# Autodesk Inventor assembly: mill_assembly
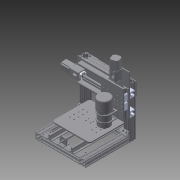
[picture p0: Inventor's stored thumbnail of the model, 180x180]
Saved by Autodesk Inventor 2014 (Build 180170000, 170)
## iProperties
Created: 2014-08-08
Part Number: mill_assembly
Document SubType Name: Assembly
Designer: Matthew
Author: Matthew
## Documents named in this file (29)
- C:\Users\Matthew\Documents\GitHub\CNC Mill\mill_assembly.iam
- C:\Users\Matthew\Documents\GitHub\CNC Mill\Imported Components\8020-2040\Assembly2.iam
- C:\Users\Matthew\Documents\GitHub\CNC Mill\8020\2020.ipt
- C:\Users\Matthew\Documents\GitHub\CNC Mill\8020\2020_18in.ipt
- C:\Users\Matthew\Documents\GitHub\CNC Mill\plate_4127.ipt
- C:\Users\Matthew\Documents\GitHub\CNC Mill\8020\gusset_4138.ipt
- C:\Users\Matthew\Documents\GitHub\CNC Mill\8020\gusset_4134.ipt
- C:\Users\Matthew\Documents\GitHub\CNC Mill\mic6_plate.ipt
- C:\Users\Matthew\Documents\GitHub\CNC Mill\1605\1605_400mm.ipt
- C:\Users\Matthew\Documents\GitHub\CNC Mill\1605\1605_ballnut.ipt
- C:\Users\Matthew\Documents\GitHub\CNC Mill\y_axis_mounting_plate.ipt
- C:\Users\Matthew\Documents\GitHub\CNC Mill\nema23_motor_mount.ipt
- C:\Users\Matthew\Documents\GitHub\CNC Mill\fk12.ipt
- C:\Users\Matthew\Documents\GitHub\CNC Mill\sbr\sbr20\SBR20UU.iam
- C:\Users\Matthew\Documents\GitHub\CNC Mill\6.35x10mm_coupler.ipt
- C:\Users\Matthew\Documents\GitHub\CNC Mill\sbr\sbr20\sbr20_400mm.ipt
- C:\Users\Matthew\Documents\GitHub\CNC Mill\HD16.ipt
- C:\Users\Matthew\Documents\GitHub\CNC Mill\nema23_HS8630.ipt
- C:\Users\Matthew\Documents\GitHub\CNC Mill\sbr\sbr20\sbr20_210mm.ipt
- C:\Users\Matthew\Documents\GitHub\CNC Mill\sbr\sbr20\sbr20_360mm.ipt
- C:\Users\Matthew\Documents\GitHub\CNC Mill\z-axis_mount_plate.ipt
- C:\Users\Matthew\Documents\GitHub\CNC Mill\1605\1605_200mm.ipt
- C:\Users\Matthew\Documents\GitHub\CNC Mill\y-axis_mount_plate.ipt
- C:\Users\Matthew\Documents\GitHub\CNC Mill\8020\2020_16in.ipt
- C:\Users\Matthew\Documents\GitHub\CNC Mill\router_plate.ipt
- C:\Users\Matthew\Documents\GitHub\CNC Mill\router_mount.ipt
- C:\Users\Matthew\Documents\GitHub\CNC Mill\1617evs.ipt
- C:\Users\Matthew\Documents\GitHub\CNC Mill\ff12_mount.ipt
- C:\Users\Matthew\Documents\GitHub\CNC Mill\ff12.ipt
## Components (67 placed, 28 different names)
1. Assembly2:1 [sub-assembly] — Mate:22, Mate:24, Mate:26, Mate:39, Mate:41, Mate:42, Mate:43, Mate:45, Mate:161, Flush:91, Flush:114, Flush:115, Mate:184, Flush:117, Flush:118, Mate:185
2. 2020_18in:1 — Mate:31, Mate:32, Mate:38, Mate:47, Mate:48, Mate:111, Flush:66, Mate:181, Flush:107, Flush:108, Flush:113
3. 2020_18in:2 — Mate:28, Mate:29, Mate:34, Mate:50, Mate:51, Flush:60, Flush:109, Flush:110, Mate:182
4. 2020:3 — Mate:46, Mate:49, Mate:115, Flush:63, Mate:116, Mate:127, Mate:128, Flush:111, Flush:112, Mate:183
5. 2020:4 — Mate:111, Flush:60, Mate:113, Mate:114, Flush:66, Flush:67, Flush:68, Flush:108, Flush:109, Flush:110, Mate:182, Flush:124, Mate:190
6. plate_4127:1 — Mate:39, Mate:41, Flush:119
7. gusset_4138:1 — Mate:22
8. gusset_4134:1 — Mate:28, Mate:29
9. gusset_4138:2 — Mate:24, Mate:26
10. gusset_4134:2 — Mate:31, Mate:32
11. gusset_4134:3 — Mate:34, Mate:113, Flush:61
12. gusset_4134:4 — Mate:38, Mate:114, Flush:62
13. plate_4127:2 — Mate:42, Mate:43, Mate:45, Flush:116
14. gusset_4134:5 — Mate:49, Mate:50, Mate:51
15. gusset_4134:6 — Mate:46, Mate:47, Mate:48, Flush:61, Flush:62
16. mic6_plate:1 — Flush:76, Flush:77, Mate:141
17. 1605_400mm:1 — Mate:98, Mate:100, Mate:108, Insert:2
18. 1605_ballnut:1 — Mate:108, Mate:133, Mate:134, Flush:75
19. y_axis_mounting_plate:1
20. nema23_motor_mount:1 — Mate:99, Mate:115, Flush:63, Mate:116, Mate:136, Mate:137
21. nema23_motor_mount:2 — Mate:153, Flush:86, Mate:154, Mate:155, Mate:156, Mate:157
22. 1605_ballnut:5
23. 1605_ballnut:6 — Mate:150, Mate:158, Flush:90, Mate:159
24. fk12:1 — Mate:98, Mate:99, Mate:100, Mate:137
25. nema23_motor_mount:3
26. fk12:3 — Mate:156, Mate:157
27. SBR20UU:1 [sub-assembly] — Mate:131, Flush:69, Flush:70, Flush:73, Mate:138, Mate:140, Flush:77, Mate:141
28. 6.35x10mm_coupler:1 — Insert:3, Insert:4
29. sbr20_400mm:1 — Mate:127, Flush:67, Mate:130
30. SBR20UU:2 [sub-assembly] — Mate:129, Mate:132, Flush:71, Flush:72, Mate:139
31. sbr20_400mm:2 — Flush:68, Mate:128, Mate:129
32. SBR20UU:3 [sub-assembly] — Mate:130, Mate:131, Flush:69, Flush:70, Flush:74, Flush:76
33. SBR20UU:4 [sub-assembly] — Mate:132, Flush:71, Flush:72, Flush:73, Flush:74
34. HD16:1 — Mate:133, Mate:134, Flush:75, Mate:138, Mate:139, Mate:140
35. nema23_HS8630:1 — Mate:135, Mate:136
36. 6.35x10mm_coupler:2 — Insert:2, Mate:135
37. sbr20_210mm:1 — Mate:143, Mate:149, Flush:82, Mate:168, Flush:104
38. sbr20_360mm:1 — Mate:162, Flush:92, Mate:165, Mate:178, Flush:106
39. SBR20UU:5 [sub-assembly] — Mate:143, Flush:78, Flush:79, Mate:144, Flush:84, Flush:85, Mate:160
40. SBR20UU:6 [sub-assembly] — Flush:78, Flush:79, Mate:144
41. sbr20_210mm:2 — Mate:148, Flush:83, Mate:169
42. SBR20UU:7 [sub-assembly] — Flush:84, Flush:85
43. SBR20UU:8 [sub-assembly]
44. z-axis_mount_plate:1 — Mate:148, Mate:149, Flush:82, Flush:83, Mate:153, Flush:86, Mate:167, Flush:102, Flush:103, Flush:104
45. 1605_200mm:1 — Mate:150, Insert:3
46. nema23_HS8630:2 — Mate:154, Mate:155, Insert:4
47. HD16:6 — Mate:158, Flush:90, Mate:159, Mate:160, Mate:168, Mate:169, Mate:186, Flush:120, Flush:121
48. y-axis_mount_plate:1 — Mate:161, Flush:91, Mate:162, Mate:163, Mate:177, Flush:106
49. sbr20_360mm:2 — Flush:92, Mate:163, Mate:164, Mate:179, Mate:188
50. SBR20UU:9 [sub-assembly] — Mate:164, Flush:95, Flush:96, Flush:99, Flush:101, Mate:167, Flush:103
51. SBR20UU:10 [sub-assembly] — Mate:165, Flush:95, Flush:96, Mate:166, Flush:97, Flush:98, Flush:102
52. SBR20UU:11 [sub-assembly] — Flush:99, Flush:100, Flush:101
53. SBR20UU:12 [sub-assembly] — Mate:166, Flush:97, Flush:98, Flush:100, Mate:180
54. nema23_motor_mount:4 — Mate:177
55. fk12:4 — Insert:8, Mate:188
56. 6.35x10mm_coupler:3
57. nema23_HS8630:3
58. 1605_400mm:2 — Mate:176, Insert:8
59. 1605_ballnut:7 — Mate:176
60. HD16:7 — Mate:178, Mate:179, Mate:180
61. 2020_16in:1 — Mate:181, Flush:107, Flush:111, Flush:112, Flush:113, Mate:183, Flush:114, Flush:115, Mate:184, Flush:116
62. 2020_16in:2 — Flush:117, Flush:118, Mate:185, Flush:119
63. router_plate:1 — Mate:186, Flush:120, Flush:121, Mate:187, Flush:122, Flush:123
64. router_mount:1 — Insert:7, Mate:187, Flush:122, Flush:123
65. 1617evs:1 — Insert:7
66. ff12_mount:1 — Flush:124, Mate:190, Insert:9
67. ff12:1 — Insert:9
## Relationships (153: Mate 88, Flush 58, Insert 7)
- Mate:22: Assembly2:1 ↔ gusset_4138:1
- Mate:24: Assembly2:1 ↔ gusset_4138:2
- Mate:26: Assembly2:1 ↔ gusset_4138:2
- Mate:28: 2020_18in:2 ↔ gusset_4134:1
- Mate:29: 2020_18in:2 ↔ gusset_4134:1
- Mate:31: 2020_18in:1 ↔ gusset_4134:2
- Mate:32: 2020_18in:1 ↔ gusset_4134:2
- Mate:34: 2020_18in:2 ↔ gusset_4134:3
- Mate:38: 2020_18in:1 ↔ gusset_4134:4
- Mate:39: Assembly2:1 ↔ plate_4127:1
- Mate:41: Assembly2:1 ↔ plate_4127:1
- Mate:42: Assembly2:1 ↔ plate_4127:2
- Mate:43: Assembly2:1 ↔ plate_4127:2
- Mate:45: Assembly2:1 ↔ plate_4127:2
- Mate:46: 2020:3 ↔ gusset_4134:6
- Mate:47: 2020_18in:1 ↔ gusset_4134:6
- Mate:48: 2020_18in:1 ↔ gusset_4134:6
- Mate:49: 2020:3 ↔ gusset_4134:5
- Mate:50: 2020_18in:2 ↔ gusset_4134:5
- Mate:51: 2020_18in:2 ↔ gusset_4134:5
- Mate:98: 1605_400mm:1 ↔ fk12:1
- Mate:99: nema23_motor_mount:1 ↔ fk12:1
- Mate:100: 1605_400mm:1 ↔ fk12:1
- Mate:108: 1605_400mm:1 ↔ 1605_ballnut:1
- Mate:111: 2020_18in:1 ↔ 2020:4
- Flush:60: 2020_18in:2 ↔ 2020:4
- Mate:113: 2020:4 ↔ gusset_4134:3
- Flush:61: gusset_4134:3 ↔ gusset_4134:6
- Mate:114: 2020:4 ↔ gusset_4134:4
- Flush:62: gusset_4134:4 ↔ gusset_4134:6
- Mate:115: 2020:3 ↔ nema23_motor_mount:1
- Flush:63: 2020:3 ↔ nema23_motor_mount:1
- Mate:116 (124.2695 mm): 2020:3 ↔ nema23_motor_mount:1
- Flush:66: 2020_18in:1 ↔ 2020:4
- Mate:127: 2020:3 ↔ sbr20_400mm:1
- Flush:67: 2020:4 ↔ sbr20_400mm:1
- Flush:68: 2020:4 ↔ sbr20_400mm:2
- Mate:128: 2020:3 ↔ sbr20_400mm:2
- Mate:129: SBR20UU:2 ↔ sbr20_400mm:2
- Mate:130: sbr20_400mm:1 ↔ SBR20UU:3
- Mate:131 (20 mm): SBR20UU:1 ↔ SBR20UU:3
- Flush:69: SBR20UU:1 ↔ SBR20UU:3
- Flush:70: SBR20UU:1 ↔ SBR20UU:3
- Mate:132 (20 mm): SBR20UU:2 ↔ SBR20UU:4
- Flush:71: SBR20UU:2 ↔ SBR20UU:4
- Flush:72: SBR20UU:2 ↔ SBR20UU:4
- Flush:73: SBR20UU:1 ↔ SBR20UU:4
- Flush:74: SBR20UU:3 ↔ SBR20UU:4
- Mate:133: 1605_ballnut:1 ↔ HD16:1
- Mate:134: 1605_ballnut:1 ↔ HD16:1
- Flush:75: 1605_ballnut:1 ↔ HD16:1
- Insert:2 (-12.5 mm): 1605_400mm:1 ↔ 6.35x10mm_coupler:2
- Mate:135: nema23_HS8630:1 ↔ 6.35x10mm_coupler:2
- Mate:136: nema23_motor_mount:1 ↔ nema23_HS8630:1
- Mate:137: nema23_motor_mount:1 ↔ fk12:1
- Mate:138 (42.3 mm): SBR20UU:1 ↔ HD16:1
- Mate:139 (42.3 mm): SBR20UU:2 ↔ HD16:1
- Mate:140 (-7.5 mm): SBR20UU:1 ↔ HD16:1
- Flush:76 (38.1 mm): mic6_plate:1 ↔ SBR20UU:3
- Flush:77 (-92.4052 mm): mic6_plate:1 ↔ SBR20UU:1
- Mate:141: mic6_plate:1 ↔ SBR20UU:1
- Mate:143: sbr20_210mm:1 ↔ SBR20UU:5
- Flush:78: SBR20UU:5 ↔ SBR20UU:6
- Flush:79: SBR20UU:5 ↔ SBR20UU:6
- Mate:144 (10 mm): SBR20UU:5 ↔ SBR20UU:6
- [Mate]: sbr20_210mm:2 ↔ SBR20UU:7
- [Flush]: SBR20UU:7 ↔ SBR20UU:8
- [Flush]: SBR20UU:7 ↔ SBR20UU:8
- [Mate] (10 mm): SBR20UU:7 ↔ SBR20UU:8
- Mate:148: sbr20_210mm:2 ↔ z-axis_mount_plate:1
- Mate:149: sbr20_210mm:1 ↔ z-axis_mount_plate:1
- Flush:82: sbr20_210mm:1 ↔ z-axis_mount_plate:1
- Flush:83: sbr20_210mm:2 ↔ z-axis_mount_plate:1
- Flush:84: SBR20UU:5 ↔ SBR20UU:7
- Flush:85: SBR20UU:5 ↔ SBR20UU:7
- Mate:150: 1605_ballnut:6 ↔ 1605_200mm:1
- Insert:3 (-12.5 mm): 6.35x10mm_coupler:1 ↔ 1605_200mm:1
- Mate:153: nema23_motor_mount:2 ↔ z-axis_mount_plate:1
- Flush:86: nema23_motor_mount:2 ↔ z-axis_mount_plate:1
- Mate:154: nema23_motor_mount:2 ↔ nema23_HS8630:2
- Mate:155: nema23_motor_mount:2 ↔ nema23_HS8630:2
- Insert:4 (-7 mm): 6.35x10mm_coupler:1 ↔ nema23_HS8630:2
- Mate:156: nema23_motor_mount:2 ↔ fk12:3
- Mate:157: nema23_motor_mount:2 ↔ fk12:3
- Mate:158: 1605_ballnut:6 ↔ HD16:6
- Flush:90: 1605_ballnut:6 ↔ HD16:6
- Mate:159: 1605_ballnut:6 ↔ HD16:6
- Mate:160 (-12.5 mm): SBR20UU:5 ↔ HD16:6
- Mate:161: Assembly2:1 ↔ y-axis_mount_plate:1
- Flush:91: Assembly2:1 ↔ y-axis_mount_plate:1
- Mate:162: sbr20_360mm:1 ↔ y-axis_mount_plate:1
- Flush:92: sbr20_360mm:1 ↔ sbr20_360mm:2
- Mate:163: y-axis_mount_plate:1 ↔ sbr20_360mm:2
- Mate:164: sbr20_360mm:2 ↔ SBR20UU:9
- Mate:165: sbr20_360mm:1 ↔ SBR20UU:10
- Flush:95: SBR20UU:9 ↔ SBR20UU:10
- Flush:96: SBR20UU:9 ↔ SBR20UU:10
- Mate:166 (60 mm): SBR20UU:10 ↔ SBR20UU:12
- Flush:97: SBR20UU:10 ↔ SBR20UU:12
- Flush:98: SBR20UU:10 ↔ SBR20UU:12
- Flush:99: SBR20UU:9 ↔ SBR20UU:11
- Flush:100: SBR20UU:11 ↔ SBR20UU:12
- Flush:101: SBR20UU:9 ↔ SBR20UU:11
- Mate:167: z-axis_mount_plate:1 ↔ SBR20UU:9
- Flush:102: z-axis_mount_plate:1 ↔ SBR20UU:10
- Flush:103: z-axis_mount_plate:1 ↔ SBR20UU:9
- Mate:168 (11 mm): sbr20_210mm:1 ↔ HD16:6
- Mate:169 (11 mm): sbr20_210mm:2 ↔ HD16:6
- Flush:104: sbr20_210mm:1 ↔ z-axis_mount_plate:1
- [Mate]: nema23_motor_mount:4 ↔ nema23_HS8630:3
- [Mate]: nema23_motor_mount:4 ↔ nema23_HS8630:3
- [Insert] (-7 mm): 6.35x10mm_coupler:3 ↔ nema23_HS8630:3
- [Mate]: nema23_motor_mount:4 ↔ fk12:4
- [Mate]: nema23_motor_mount:4 ↔ fk12:4
- [Mate]: 1605_ballnut:7 ↔ HD16:7
- [Flush]: 1605_ballnut:7 ↔ HD16:7
- [Mate]: 1605_ballnut:7 ↔ HD16:7
- Mate:176: 1605_400mm:2 ↔ 1605_ballnut:7
- Mate:177: y-axis_mount_plate:1 ↔ nema23_motor_mount:4
- Mate:178 (19.9 mm): sbr20_360mm:1 ↔ HD16:7
- Mate:179 (19.9 mm): sbr20_360mm:2 ↔ HD16:7
- Flush:106: sbr20_360mm:1 ↔ y-axis_mount_plate:1
- Mate:180 (12.5 mm): SBR20UU:12 ↔ HD16:7
- Mate:181: 2020_18in:1 ↔ 2020_16in:1
- Flush:107: 2020_18in:1 ↔ 2020_16in:1
- Flush:108: 2020_18in:1 ↔ 2020:4
- Flush:109: 2020_18in:2 ↔ 2020:4
- Flush:110: 2020_18in:2 ↔ 2020:4
- Mate:182: 2020_18in:2 ↔ 2020:4
- Flush:111: 2020:3 ↔ 2020_16in:1
- Flush:112: 2020:3 ↔ 2020_16in:1
- Flush:113: 2020_18in:1 ↔ 2020_16in:1
- Mate:183: 2020:3 ↔ 2020_16in:1
- Flush:114: Assembly2:1 ↔ 2020_16in:1
- Flush:115: Assembly2:1 ↔ 2020_16in:1
- Mate:184: Assembly2:1 ↔ 2020_16in:1
- Flush:116: plate_4127:2 ↔ 2020_16in:1
- Flush:117: Assembly2:1 ↔ 2020_16in:2
- Flush:118: Assembly2:1 ↔ 2020_16in:2
- Mate:185: Assembly2:1 ↔ 2020_16in:2
- Flush:119: plate_4127:1 ↔ 2020_16in:2
- Insert:7: router_mount:1 ↔ 1617evs:1
- Mate:186: HD16:6 ↔ router_plate:1
- Flush:120 (-96.7994 mm): HD16:6 ↔ router_plate:1
- Flush:121 (64.897 mm): HD16:6 ↔ router_plate:1
- Mate:187: router_plate:1 ↔ router_mount:1
- Flush:122: router_plate:1 ↔ router_mount:1
- Flush:123 (44.45 mm): router_plate:1 ↔ router_mount:1
- Insert:8: fk12:4 ↔ 1605_400mm:2
- Mate:188 (-40 mm): sbr20_360mm:2 ↔ fk12:4
- Flush:124: 2020:4 ↔ ff12_mount:1
- Mate:190: 2020:4 ↔ ff12_mount:1
- Insert:9: ff12_mount:1 ↔ ff12:1
## Named parameters: mountspace = 20 mm, yoffset = 42.3 mm, d321_d318 = 0 mm, d322_d319 = 0 mm, d323_d320 = 10 mm, d324_d317 = 0 mm, yaxisspacing = 60 mm, zaxissbrspacing = 11 mm, d373_d340 = -7 mm, d374_d341 = 0 mm, d375_d342 = 0 mm, d376_d338 = 0 mm, d377_d339 = 0 mm, d379_d346 = 0 mm, d380_d347 = 0 mm, d381_d348 = 0 mm, yaxissbrspacing = 19.9 mm
